# Autodesk Inventor assembly: rotor
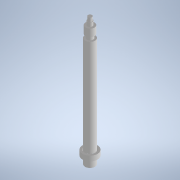
[picture p0: Inventor's stored thumbnail of the model, 180x180]
Saved by Autodesk Inventor 2021 (Build 250183000, 183)
## iProperties
Created: 2020-12-17
Part Number: rotor
Document SubType Name: Assembly
Designer: Yuri
Author: Yuri
## Documents named in this file (5)
- C:\Users\Yuri\Documents\MATLAB\save\rotor_model\rotor.iam
- C:\Users\Yuri\YandexDisk\Учеба\ВКР\Расчет подшипника\model_beering\invertor\n_rotor\ber.ipt
- C:\Users\Yuri\YandexDisk\Учеба\ВКР\Расчет подшипника\model_beering\invertor\n_rotor\muft.ipt
- C:\Users\Yuri\YandexDisk\Учеба\ВКР\Расчет подшипника\model_beering\invertor\n_rotor\val.ipt
- C:\Users\Yuri\YandexDisk\Учеба\ВКР\Расчет подшипника\model_beering\invertor\n_rotor\val_rot.ipt
## Components (4 placed, 4 different names)
1. ber:1 — Цилиндрический:1
2. muft:1 — Цилиндрический:2, Вставка:1, Цилиндрический:3
3. val:1 — Цилиндрический:1, Цилиндрический:2, Вставка:1
4. val_rot:1 — Цилиндрический:3
## Relationships (4: CylindricalJoint 3, Insert 1)
- Цилиндрический:1 [CylindricalJoint]: ber:1 ↔ val:1
- Цилиндрический:2 [CylindricalJoint]: muft:1 ↔ val:1
- Вставка:1 [Insert] (15 mm): muft:1 ↔ val:1
- Цилиндрический:3 [CylindricalJoint]: muft:1 ↔ val_rot:1
